# Autodesk Inventor assembly: 1410-03-10 Carte laser
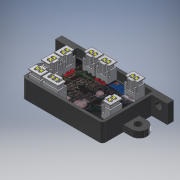
[picture p0: Inventor's stored thumbnail of the model, 180x180]
Saved by Autodesk Inventor 2017 (Build 210142000, 142)
## iProperties
Part Number: 1410-03-10 Carte laser
Material: Générique
Document SubType Name: Assembly
Designer: Adrien MARY
Author: Adrien MARY
## Documents named in this file (5)
- W:\Professionnel\Conception FABLAB\1410-LaserShow\1410-03 Composant electronique\1410-03-10 Carte laser.iam
- W:\Professionnel\Conception FABLAB\1410-LaserShow\1410-03 Composant electronique\1410-03-01 Carte electronique laser.ipt
- W:\Professionnel\Conception FABLAB\1410-LaserShow\1410-04 Connecteur_JST\Connecteur_JST\Connecteur jst 2 broches.iam
- W:\Professionnel\Conception FABLAB\1410-LaserShow\1410-04 Connecteur_JST\Connecteur_JST.iam
- W:\Professionnel\Conception FABLAB\1410-LaserShow\1410-04 Connecteur_JST\Connecteur_JST\Connecteur jst 3 broches.iam
## Components (9 placed, 3 different names)
1. Carte_laser:1 — Placage:1, Placage:2, Placage:3, Placage:4, Placage:5, Placage:6, Placage:7, Placage:8, Placage:10, Placage:12, Placage:13, Placage:14, Placage:15, Placage:16, Placage:17
2. Connecteur jst 2 broches:1 [sub-assembly] — Affleurement:3, Affleurement:4, Placage:1, Placage:3, Placage:9, Placage:10
3. Connecteur jst 2 broches:2 [sub-assembly] — Affleurement:2, Placage:7, Placage:14
4. Connecteur jst 2 broches:3 [sub-assembly] — Affleurement:1, Placage:8, Placage:15
5. Connecteur jst 2 broches:4 [sub-assembly] — Affleurement:6, Placage:4, Placage:11, Placage:12
6. Connecteur jst 2 broches:5 [sub-assembly] — Affleurement:5, Affleurement:6, Placage:5, Placage:11
7. Connecteur jst 2 broches:6 [sub-assembly] — Affleurement:4, Affleurement:5, Placage:2, Placage:9
8. Connecteur jst 2 broches:7 [sub-assembly] — Affleurement:1, Affleurement:2, Affleurement:3, Placage:6, Placage:13, Placage:18
9. Connecteur jst 3 broches:8 [sub-assembly] — Placage:16, Placage:17, Placage:18
## Relationships (24: Mate 18, Flush 6)
- Affleurement:1 [Flush]: Connecteur jst 2 broches:3 ↔ Connecteur jst 2 broches:7
- Affleurement:2 [Flush]: Connecteur jst 2 broches:2 ↔ Connecteur jst 2 broches:7
- Affleurement:3 [Flush]: Connecteur jst 2 broches:1 ↔ Connecteur jst 2 broches:7
- Affleurement:4 [Flush]: Connecteur jst 2 broches:1 ↔ Connecteur jst 2 broches:6
- Affleurement:5 [Flush]: Connecteur jst 2 broches:5 ↔ Connecteur jst 2 broches:6
- Affleurement:6 [Flush]: Connecteur jst 2 broches:4 ↔ Connecteur jst 2 broches:5
- Placage:1 [Mate]: Carte_laser:1 ↔ Connecteur jst 2 broches:1
- Placage:2 [Mate]: Carte_laser:1 ↔ Connecteur jst 2 broches:6
- Placage:3 [Mate]: Carte_laser:1 ↔ Connecteur jst 2 broches:1
- Placage:4 [Mate]: Carte_laser:1 ↔ Connecteur jst 2 broches:4
- Placage:5 [Mate]: Carte_laser:1 ↔ Connecteur jst 2 broches:5
- Placage:6 [Mate]: Carte_laser:1 ↔ Connecteur jst 2 broches:7
- Placage:7 [Mate]: Carte_laser:1 ↔ Connecteur jst 2 broches:2
- Placage:8 [Mate] (1 mm): Carte_laser:1 ↔ Connecteur jst 2 broches:3
- Placage:9 [Mate] (1 mm): Connecteur jst 2 broches:1 ↔ Connecteur jst 2 broches:6
- Placage:10 [Mate] (9 mm): Carte_laser:1 ↔ Connecteur jst 2 broches:1
- Placage:11 [Mate] (1 mm): Connecteur jst 2 broches:4 ↔ Connecteur jst 2 broches:5
- Placage:12 [Mate] (7 mm): Carte_laser:1 ↔ Connecteur jst 2 broches:4
- Placage:13 [Mate] (1 mm): Carte_laser:1 ↔ Connecteur jst 2 broches:7
- Placage:14 [Mate] (5 mm): Carte_laser:1 ↔ Connecteur jst 2 broches:2
- Placage:15 [Mate] (6 mm): Carte_laser:1 ↔ Connecteur jst 2 broches:3
- Placage:16 [Mate]: Carte_laser:1 ↔ Connecteur jst 3 broches:8
- Placage:17 [Mate]: Carte_laser:1 ↔ Connecteur jst 3 broches:8
- Placage:18 [Mate] (1 mm): Connecteur jst 2 broches:7 ↔ Connecteur jst 3 broches:8
